# Autodesk Inventor assembly: ASY NDM_VOS pillar 1
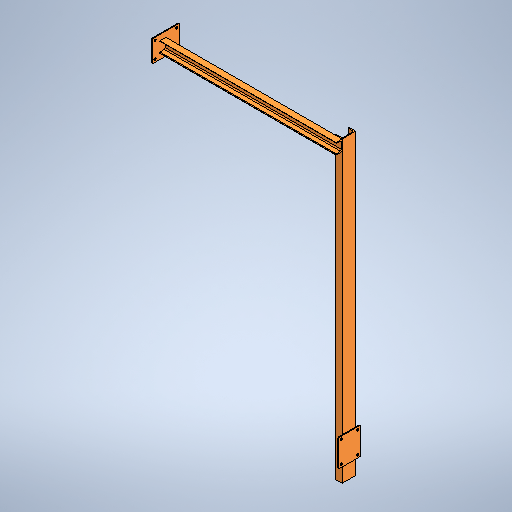
[picture p0: Inventor's stored thumbnail of the model, 512x512]
Saved by Autodesk Inventor 2025 (Build 290162010, 162A)
## iProperties
Created: 2025-11-03
Part Number: ASY NDM_VOS pillar 1
Document SubType Name: Assembly
Designer: admin
Mass: 33702.5 g
Surface Area: 13636.4 cm^2
Volume: 4619.65 cm^3
Density: 7.29547 g/cm^3
Author: admin
## Documents named in this file (4)
- C:\Users\admin\Yandex.Disk\home pc\Inventor\NDM-VOS_powder_hopper\400 tube\ASY NDM_VOS pillar 1.iam
- C:\Users\admin\Yandex.Disk\home pc\Inventor\NDM-VOS_powder_hopper\400 tube\NDM-VOS pillar 1 ch 1.ipt
- C:\Users\admin\Yandex.Disk\home pc\Inventor\NDM-VOS_powder_hopper\400 tube\Part2.ipt
- C:\Users\admin\Yandex.Disk\home pc\Inventor\NDM-VOS_powder_hopper\400 tube\NDM-VOS pillar 1 ch 2.ipt
## Components (4 placed, 3 different names)
1. NDM-VOS pillar 1 ch 1:1 — Rigid:1, Mate:1, Mate:2, Rigid:2
2. Part2:1 — Rigid:1, Flush:1
3. NDM-VOS pillar 1 ch 2:1 — Rigid:2, Rigid:3
4. Part2:2 — Rigid:3
## Relationships (6: WeldJoint 3, Mate 2, Flush 1)
- Rigid:1 [WeldJoint] (110 mm): NDM-VOS pillar 1 ch 1:1 ↔ Part2:1
- Mate:1: NDM-VOS pillar 1 ch 1:1
- Flush:1: Part2:1
- Mate:2: NDM-VOS pillar 1 ch 1:1
- Rigid:2 [WeldJoint]: NDM-VOS pillar 1 ch 1:1 ↔ NDM-VOS pillar 1 ch 2:1
- Rigid:3 [WeldJoint]: NDM-VOS pillar 1 ch 2:1 ↔ Part2:2
